# Autodesk Inventor assembly: Chassis and wheels assembly
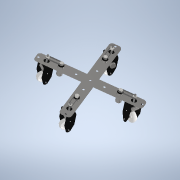
[picture p0: Inventor's stored thumbnail of the model, 180x180]
Saved by Autodesk Inventor 2020.3 (Build 243373000, 373)
## iProperties
Created: 2022-07-01
Part Number: Chassis and wheels assembly
Document SubType Name: Assembly
Designer: karimi2
Author: karimi2
## Documents named in this file (8)
- C:\Users\Public\D\Desktop\mechanicalDesign\src\Chassis and wheels assembly.iam
- C:\Users\Public\D\Desktop\mechanicalDesign\src\chassisPart1.ipt
- C:\Users\Public\D\Desktop\mechanicalDesign\src\GearedDCmotor.ipt
- C:\Users\Public\D\Desktop\mechanicalDesign\src\Wheel Assembly.iam
- C:\Users\Public\D\Desktop\mechanicalDesign\src\Chassis and wheels assembly\Design Accelerator\Synchronous Belts Transmission2.iam
- C:\Users\Public\D\Desktop\mechanicalDesign\src\Chassis and wheels assembly\Design Accelerator\Synchronous Belts Transmission3.iam
- C:\Users\Public\D\Desktop\mechanicalDesign\src\Chassis and wheels assembly\Design Accelerator\Synchronous Belts Transmission4.iam
- C:\Users\Public\D\Desktop\mechanicalDesign\src\Chassis and wheels assembly\Design Accelerator\Synchronous Belts Transmission5.iam
## Components (14 placed, 4 different names)
1. chassisPart1:1 — Rigid:1, Rigid:2, Rigid:3, Rigid:4, Rigid:6, Rigid:7
2. chassisPart1:2 — Rigid:1, Rotational:2, Rigid:5, Rigid:8, Rigid:9
3. GearedDCmotor:1 — Rigid:2, Mate:1
4. Wheel Assembly:1 [sub-assembly] — Rigid:3, Rigid:4, Rotational:1
5. Synchronous Belts Transmission:1 [sub-assembly] — Rotational:1, Mate:1
6. Wheel Assembly:2 [sub-assembly] — Rotational:2
7. GearedDCmotor:2 — Rigid:5
8. Synchronous Belts Transmission:2 [sub-assembly]
9. Wheel Assembly:3 [sub-assembly] — Rigid:6
10. GearedDCmotor:3 — Rigid:7
11. Synchronous Belts Transmission:3 [sub-assembly]
12. Wheel Assembly:4 [sub-assembly] — Rigid:8, Mate:3, Flush:1
13. GearedDCmotor:4 — Rigid:9, Mate:2
14. Synchronous Belts Transmission:4 [sub-assembly] — Mate:2, Mate:3, Flush:1
## Relationships (15: WeldJoint 9, Mate 3, RevoluteJoint 2, Flush 1)
- Rigid:1 [WeldJoint] (2 mm): chassisPart1:1 ↔ chassisPart1:2
- Rigid:2 [WeldJoint]: chassisPart1:1 ↔ GearedDCmotor:1
- Rigid:3 [WeldJoint] (4.5 mm): chassisPart1:1 ↔ Wheel Assembly:1
- Rigid:4 [WeldJoint] (3.5 mm): chassisPart1:1 ↔ Wheel Assembly:1
- Rotational:1 [RevoluteJoint] (10 mm): Wheel Assembly:1 ↔ Synchronous Belts Transmission:1
- Mate:1: GearedDCmotor:1 ↔ Synchronous Belts Transmission:1
- Rotational:2 [RevoluteJoint]: chassisPart1:2 ↔ Wheel Assembly:2
- Rigid:5 [WeldJoint] (-10.375 mm): chassisPart1:2 ↔ GearedDCmotor:2
- Rigid:6 [WeldJoint] (-3.5 mm): chassisPart1:1 ↔ Wheel Assembly:3
- Rigid:7 [WeldJoint] (-10.375 mm): chassisPart1:1 ↔ GearedDCmotor:3
- Rigid:8 [WeldJoint] (-0.5 mm): chassisPart1:2 ↔ Wheel Assembly:4
- Rigid:9 [WeldJoint] (-10.375 mm): chassisPart1:2 ↔ GearedDCmotor:4
- Mate:2: GearedDCmotor:4 ↔ Synchronous Belts Transmission:4
- Mate:3: Wheel Assembly:4 ↔ Synchronous Belts Transmission:4
- Flush:1 (8 mm): Wheel Assembly:4 ↔ Synchronous Belts Transmission:4
